# Autodesk Inventor assembly: 組合1
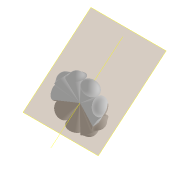
[picture p0: Inventor's stored thumbnail of the model, 180x180]
Saved by Autodesk Inventor 2022 (Build 260153000, 153)
## iProperties
Created: 2023-10-13
Part Number: 組合1
Document SubType Name: Assembly
Designer: JOU
Author: JOU
## Documents named in this file (2)
- C:\Users\JOU\Desktop\git\Special-project\接觸解析器練習資料夾\接觸解析器練習資料夾\Cycloidal Gear\ball\TEST\組合1.iam
- C:\Users\JOU\Desktop\git\Special-project\接觸解析器練習資料夾\接觸解析器練習資料夾\Cycloidal Gear\ball\TEST\錐.ipt
## Components (9 placed, 1 different names)
1. 錐:1
2. 錐:2
3. 錐:3
4. 錐:4
5. 錐:5
6. 錐:6
7. 錐:7
8. 錐:8
9. 錐:9
## Component patterns: (9 elements, first: 錐:1)
## Relationships (4: Mate 3, Angle 1)
- 貼合:1 [Mate]
- 角度:1 [Angle] (40 deg)
- 貼合:2 [Mate]
- 貼合:3 [Mate]
